# Autodesk Inventor assembly: linkage_system_test
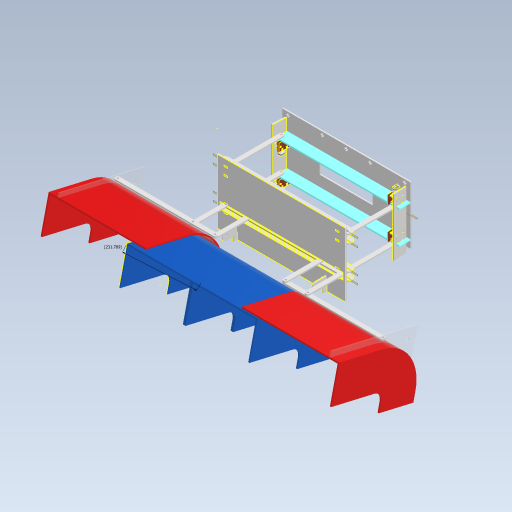
[picture p0: Inventor's stored thumbnail of the model, 512x512]
Saved by Autodesk Inventor 2023 (Build 270158000, 158)
## iProperties
Created: 2023-05-05
Part Number: linkage_system_test
Document SubType Name: Assembly
Designer: 陳詩穎
Author: 陳詩穎
## Documents named in this file (19)
- C:\Users\Johnny Jou\Documents\GitHub\Areo_Rider_Cabin\Expansion\test\linkage_system_test.iam
- C:\Users\Johnny Jou\Documents\GitHub\Areo_Rider_Cabin\Expansion\test\plate_expansion.ipt
- C:\Users\Johnny Jou\Documents\GitHub\Areo_Rider_Cabin\Expansion\test\零件1.ipt
- C:\Users\Johnny Jou\Documents\GitHub\Areo_Rider_Cabin\Expansion\test\零件4.ipt
- C:\Users\Johnny Jou\Documents\GitHub\Areo_Rider_Cabin\Expansion\test\零件5.ipt
- C:\Users\Johnny Jou\Documents\GitHub\Areo_Rider_Cabin\Expansion\test\零件7.ipt
- C:\Users\Johnny Jou\Documents\GitHub\Areo_Rider_Cabin\Airfoil & Nuzzle\nuzzle\nuzzle_v2_0327.ipt
- C:\Users\Johnny Jou\Documents\GitHub\Areo_Rider_Cabin\Airfoil & Nuzzle\nuzzle\nuzzle_v2_0516.ipt
- C:\Users\Johnny Jou\Documents\GitHub\Areo_Rider_Cabin\Airfoil & Nuzzle\nuzzle\nuzzle_v2_0516_2.ipt
- C:\Users\Johnny Jou\Documents\GitHub\Areo_Rider_Cabin\Expansion\test\零件8.ipt
- C:\Users\Johnny Jou\Documents\GitHub\Areo_Rider_Cabin\Expansion\test\零件9.ipt
- C:\Users\Johnny Jou\Documents\GitHub\Areo_Rider_Cabin\Expansion\test\零件10.ipt
- C:\Users\Johnny Jou\Documents\GitHub\Areo_Rider_Cabin\Expansion\test\零件12.ipt
- C:\Users\Johnny Jou\Documents\GitHub\Areo_Rider_Cabin\car\motor.iam
- C:\Users\Johnny Jou\Documents\GitHub\Areo_Rider_Cabin\Expansion\test\adjustable_130.ipt
- C:\Users\Johnny Jou\Documents\GitHub\Areo_Rider_Cabin\Expansion\test\adjustable_120.ipt
- C:\Users\Johnny Jou\Documents\GitHub\Areo_Rider_Cabin\Expansion\test\adjustable_200.ipt
- C:\Users\Johnny Jou\Documents\GitHub\Areo_Rider_Cabin\Expansion\test\adjustable_80.ipt
- C:\Users\Johnny Jou\Documents\GitHub\Areo_Rider_Cabin\Expansion\test\零件13.ipt
## Components (33 placed, 18 different names)
1. plate_expansion:1 — 貼合:1, 齊平:1, 貼合:2, 齊平:2, 貼合:13, 角度:1, 角度:2, 角度:3, 齊平:13
2. 零件1:1 — 齊平:2, 貼合:13, 貼合:50, 插入:3, 插入:4, 齊平:11, 貼合:219, 貼合:224, 貼合:225, 貼合:227
3. 零件1:2 — 貼合:1, 齊平:1, 貼合:2, 貼合:49, 貼合:51, 貼合:173, 貼合:175, 貼合:176, 插入:1, 齊平:11, 貼合:222, 貼合:223, 貼合:226
4. 零件8:1 — 貼合:49, 貼合:50, 貼合:51, 貼合:172
5. motor:1 [sub-assembly] — 貼合:172, 貼合:173, 貼合:174, 齊平:20
6. adjustable_120:1 — 插入:1, 角度:2, 插入:16, 貼合:194
7. adjustable_120:2 — 貼合:174, 貼合:175, 貼合:176, 插入:14, 貼合:184
8. adjustable_200:2 — 插入:3, 插入:6, 插入:12, 貼合:179, 貼合:194, 貼合:221
9. adjustable_200:3 — 插入:4, 插入:5, 插入:9, 角度:3, 貼合:218
10. 零件12:1 — 插入:5, 插入:7, 貼合:180, 貼合:181, 貼合:182, 貼合:192
11. 零件12:2 — 插入:6, 貼合:177, 貼合:228
12. adjustable_80:2 — 插入:7, 插入:8
13. adjustable_130:1 — 插入:8, 插入:9, 齊平:12
14. adjustable_80:3 — 貼合:178, 插入:15, 貼合:228
15. adjustable_130:2 — 插入:12, 插入:15, 齊平:12
16. 零件4:1 — 貼合:177, 貼合:178, 貼合:179, 齊平:8, 齊平:9, 齊平:10, 貼合:187
17. 零件4:2 — 貼合:183, 貼合:184, 齊平:7, 齊平:8, 貼合:189
18. 零件4:3 — 貼合:180, 貼合:181, 貼合:182, 齊平:9, 貼合:188, 貼合:191
19. 零件4:4 — 齊平:7, 貼合:190, 貼合:193
20. 零件13:1 — 插入:14, 貼合:183, 貼合:192
21. 零件5:1 — 齊平:10, 貼合:187, 貼合:188, 貼合:189, 貼合:190, 貼合:191, 角度:1, 齊平:13, 齊平:17, 貼合:208, 貼合:209, 貼合:210, 貼合:211, 貼合:212, 貼合:213
22. 零件13:2 — 插入:16, 貼合:193
23. nuzzle_v2_0327:1 — 齊平:17, 貼合:200, 貼合:201
24. nuzzle_v2_0516:1 — 貼合:202, 貼合:203, 貼合:204, 貼合:205, 齊平:18
25. nuzzle_v2_0516_2:1 — 貼合:200, 貼合:201, 貼合:202, 貼合:203, 貼合:206, 齊平:19
26. 零件9:1 — 貼合:204, 貼合:205, 貼合:207, 齊平:18
27. 零件10:1 — 貼合:206, 貼合:207, 齊平:19, 貼合:214
28. 零件7:1 — 貼合:208, 貼合:209, 貼合:210, 貼合:214
29. 零件7:2 — 貼合:211, 貼合:212, 貼合:213
30. motor:2 [sub-assembly] — 貼合:218, 貼合:219, 齊平:20
31. motor:3 [sub-assembly] — 貼合:221, 齊平:22, 貼合:224, 角度:5
32. motor:4 [sub-assembly] — 貼合:222, 齊平:22, 貼合:223
33. 零件8:2 — 貼合:225, 貼合:226, 貼合:227, 角度:5
## Relationships (83: Mate 52, Flush 15, Insert 12, Angle 4)
- 貼合:1 [Mate]: plate_expansion:1 ↔ 零件1:2
- 齊平:1 [Flush]: plate_expansion:1 ↔ 零件1:2
- 貼合:2 [Mate]: plate_expansion:1 ↔ 零件1:2
- 齊平:2 [Flush]: plate_expansion:1 ↔ 零件1:1
- 貼合:13 [Mate]: plate_expansion:1 ↔ 零件1:1
- 貼合:49 [Mate]: 零件1:2 ↔ 零件8:1
- 貼合:50 [Mate]: 零件1:1 ↔ 零件8:1
- 貼合:51 [Mate]: 零件1:2 ↔ 零件8:1
- 貼合:172 [Mate]: 零件8:1 ↔ motor:1
- 貼合:173 [Mate]: 零件1:2 ↔ motor:1
- 貼合:174 [Mate]: motor:1 ↔ adjustable_120:2
- 貼合:175 [Mate]: 零件1:2 ↔ adjustable_120:2
- 貼合:176 [Mate]: 零件1:2 ↔ adjustable_120:2
- 插入:1 [Insert]: 零件1:2 ↔ adjustable_120:1
- 插入:3 [Insert]: 零件1:1 ↔ adjustable_200:2
- 插入:4 [Insert]: 零件1:1 ↔ adjustable_200:3
- 插入:5 [Insert]: adjustable_200:3 ↔ 零件12:1
- 插入:6 [Insert]: adjustable_200:2 ↔ 零件12:2
- 插入:7 [Insert]: 零件12:1 ↔ adjustable_80:2
- 插入:8 [Insert]: adjustable_80:2 ↔ adjustable_130:1
- 插入:9 [Insert]: adjustable_200:3 ↔ adjustable_130:1
- 插入:12 [Insert]: adjustable_200:2 ↔ adjustable_130:2
- 貼合:177 [Mate]: 零件12:2 ↔ 零件4:1
- 貼合:178 [Mate]: adjustable_80:3 ↔ 零件4:1
- 貼合:179 [Mate]: adjustable_200:2 ↔ 零件4:1
- 貼合:180 [Mate]: 零件12:1 ↔ 零件4:3
- 貼合:181 [Mate]: 零件12:1 ↔ 零件4:3
- 貼合:182 [Mate]: 零件12:1 ↔ 零件4:3
- 插入:14 [Insert]: adjustable_120:2 ↔ 零件13:1
- 貼合:183 [Mate]: 零件4:2 ↔ 零件13:1
- 貼合:184 [Mate]: adjustable_120:2 ↔ 零件4:2
- 齊平:7 [Flush]: 零件4:2 ↔ 零件4:4
- 齊平:8 [Flush]: 零件4:1 ↔ 零件4:2
- 齊平:9 [Flush]: 零件4:1 ↔ 零件4:3
- 齊平:10 [Flush]: 零件4:1 ↔ 零件5:1
- 貼合:187 [Mate]: 零件4:1 ↔ 零件5:1
- 貼合:188 [Mate]: 零件4:3 ↔ 零件5:1
- 貼合:189 [Mate]: 零件4:2 ↔ 零件5:1
- 貼合:190 [Mate]: 零件4:4 ↔ 零件5:1
- 貼合:191 [Mate]: 零件4:3 ↔ 零件5:1
- 貼合:192 [Mate]: 零件12:1 ↔ 零件13:1
- 角度:1 [Angle] (0 deg): plate_expansion:1 ↔ 零件5:1
- 角度:2 [Angle] (90 deg): plate_expansion:1 ↔ adjustable_120:1
- 角度:3 [Angle] (90 deg): plate_expansion:1 ↔ adjustable_200:3
- 齊平:11 [Flush]: 零件1:1 ↔ 零件1:2
- 插入:15 [Insert]: adjustable_80:3 ↔ adjustable_130:2
- 插入:16 [Insert]: adjustable_120:1 ↔ 零件13:2
- 貼合:193 [Mate]: 零件4:4 ↔ 零件13:2
- 貼合:194 [Mate]: adjustable_120:1 ↔ adjustable_200:2
- 齊平:12 [Flush]: adjustable_130:1 ↔ adjustable_130:2
- 齊平:13 [Flush]: plate_expansion:1 ↔ 零件5:1
- 齊平:17 [Flush] (-2 mm): 零件5:1 ↔ nuzzle_v2_0327:1
- 貼合:200 [Mate]: nuzzle_v2_0327:1 ↔ nuzzle_v2_0516_2:1
- 貼合:201 [Mate]: nuzzle_v2_0327:1 ↔ nuzzle_v2_0516_2:1
- 貼合:202 [Mate]: nuzzle_v2_0516:1 ↔ nuzzle_v2_0516_2:1
- 貼合:203 [Mate]: nuzzle_v2_0516:1 ↔ nuzzle_v2_0516_2:1
- 貼合:204 [Mate]: nuzzle_v2_0516:1 ↔ 零件9:1
- 貼合:205 [Mate]: nuzzle_v2_0516:1 ↔ 零件9:1
- 貼合:206 [Mate]: nuzzle_v2_0516_2:1 ↔ 零件10:1
- 貼合:207 [Mate]: 零件9:1 ↔ 零件10:1
- 齊平:18 [Flush] (-20 mm): nuzzle_v2_0516:1 ↔ 零件9:1
- 齊平:19 [Flush] (20 mm): nuzzle_v2_0516_2:1 ↔ 零件10:1
- 貼合:208 [Mate]: 零件5:1 ↔ 零件7:1
- 貼合:209 [Mate]: 零件5:1 ↔ 零件7:1
- 貼合:210 [Mate]: 零件5:1 ↔ 零件7:1
- 貼合:211 [Mate]: 零件5:1 ↔ 零件7:2
- 貼合:212 [Mate]: 零件5:1 ↔ 零件7:2
- 貼合:213 [Mate]: 零件5:1 ↔ 零件7:2
- 貼合:214 [Mate]: 零件10:1 ↔ 零件7:1
- 貼合:218 [Mate]: adjustable_200:3 ↔ motor:2
- 貼合:219 [Mate]: 零件1:1 ↔ motor:2
- 齊平:20 [Flush]: motor:1 ↔ motor:2
- [Flush]: motor:3 ↔ motor:4
- 貼合:221 [Mate]: adjustable_200:2 ↔ motor:3
- 貼合:222 [Mate]: 零件1:2 ↔ motor:4
- 齊平:22 [Flush]: motor:3 ↔ motor:4
- 貼合:223 [Mate]: 零件1:2 ↔ motor:4
- 貼合:224 [Mate]: 零件1:1 ↔ motor:3
- 貼合:225 [Mate]: 零件1:1 ↔ 零件8:2
- 貼合:226 [Mate]: 零件1:2 ↔ 零件8:2
- 貼合:227 [Mate]: 零件1:1 ↔ 零件8:2
- 角度:5 [Angle] (0 deg): motor:3 ↔ 零件8:2
- 貼合:228 [Mate]: 零件12:2 ↔ adjustable_80:3
## Named parameters: d351_d349 = 0 mm
